# Autodesk Inventor assembly: montagem
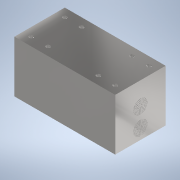
[picture p0: Inventor's stored thumbnail of the model, 180x180]
Saved by Autodesk Inventor 2021 (Build 250183000, 183)
## iProperties
Created: 2023-11-09
Part Number: montagem
Document SubType Name: Assembly
Designer: Vinicius
Author: Vinicius
## Documents named in this file (7)
- D:\Arquivos\empreendedorismo\montagem.iam
- D:\Arquivos\empreendedorismo\base-inferior.ipt
- D:\Arquivos\empreendedorismo\corpo-meio.ipt
- D:\Arquivos\empreendedorismo\suporte topo.ipt
- D:\Arquivos\empreendedorismo\placa-circuito.ipt
- D:\Arquivos\empreendedorismo\bateria.ipt
- D:\Arquivos\empreendedorismo\camera.ipt
## Components (6 placed, 6 different names)
1. base-inferior:1 — Coincidente:1, Plana:1, Coincidente:2, Coincidente:3, Coincidente:4
2. corpo-meio:1 — Plana:1, Rígida:1
3. suporte topo:1 — Rígida:1
4. placa-circuito:1 — Coincidente:2
5. bateria:1 — Coincidente:3
6. camera:1 — Coincidente:4
## Relationships (6: Mate 4, PlanarJoint 1, WeldJoint 1)
- Coincidente:1 [Mate]: base-inferior:1
- Plana:1: base-inferior:1 ↔ corpo-meio:1
- Rígida:1 [WeldJoint]: corpo-meio:1 ↔ suporte topo:1
- Coincidente:2 [Mate]: base-inferior:1 ↔ placa-circuito:1
- Coincidente:3 [Mate]: base-inferior:1 ↔ bateria:1
- Coincidente:4 [Mate]: base-inferior:1 ↔ camera:1
